# Autodesk Inventor assembly: Frame for Monitor Mounts Test
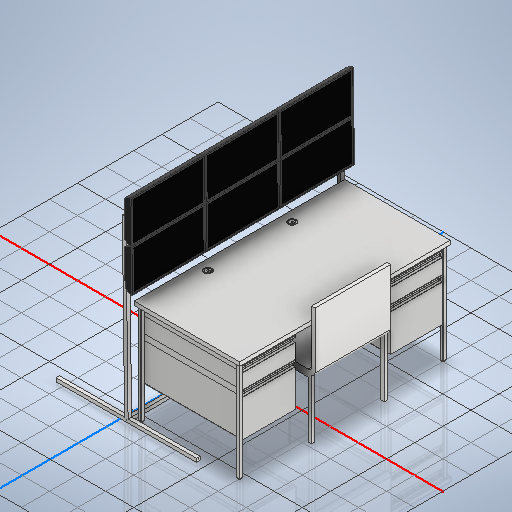
[picture p0: Inventor's stored thumbnail of the model, 512x512]
Saved by Autodesk Inventor 2027 (Build 310192000, 192)
## iProperties
Created: 2026-05-21
Part Number: Frame for Monitor Mounts Test
Document SubType Name: Assembly
Designer: IG2
Author: IG2
## Documents named in this file (8)
- C:\Users\ig2\Desktop\SMR Thermal\thermal-loop\resources\CAD_models\V0.1\Inventor\.iam files\Frame for Monitor Mounts Test.iam
- C:\Users\ig2\Downloads\Monitor v1.0.ipt
- C:\Users\ig2\Downloads\Monitor Base v1.0.ipt
- C:\Users\ig2\Downloads\Monitor Base Slide v1.0.ipt
- C:\Users\ig2\Downloads\Monitor Seat v1.0.ipt
- C:\Users\ig2\Desktop\SMR Thermal\thermal-loop\resources\CAD_models\V0.1\Inventor\.ipt files\Frame of Monitor Mount.ipt
- C:\Users\ig2\Desktop\SMR Thermal\thermal-loop\resources\CAD_models\V0.1\Inventor\.ipt files\chair.ipt
- C:\Users\ig2\Desktop\SMR Thermal\thermal-loop\resources\CAD_models\V0.1\Inventor\.ipt files\Plastic Laminate Top Desk Wide.ipt
## Components (27 placed, 7 different names)
1. Monitor v1.0:1 — Rigid:25, Rigid:32
2. Monitor v1.0:2 — Rigid:26, Rigid:29, Rigid:30
3. Monitor v1.0:3 — Rigid:24, Rigid:31, Rigid:32
4. Monitor v1.0:4 — Rigid:28, Rigid:31
5. Monitor v1.0:5 — Rigid:27, Rigid:29
6. Monitor v1.0:6 — Slider:19, Rigid:23, Rigid:30
7. Monitor Base v1.0:1 — Rotational:26
8. Monitor Base Slide v1.0:1 — Rigid:4, Rotational:26
9. Monitor Seat v1.0:1 — Rigid:1, Rigid:24, Rotational:33
10. Monitor Base v1.0:2 — Rigid:12
11. Monitor Base Slide v1.0:2 — Rigid:3, Rigid:12
12. Monitor Seat v1.0:2 — Rigid:3, Rigid:28
13. Monitor Base v1.0:3 — Rigid:2
14. Monitor Base Slide v1.0:3 — Rigid:1, Rigid:2
15. Monitor Seat v1.0:3 — Rigid:4, Rigid:25
16. Monitor Base v1.0:4 — Rigid:10
17. Monitor Base Slide v1.0:4 — Rigid:5, Rigid:10
18. Monitor Seat v1.0:4 — Rigid:5, Rigid:27
19. Monitor Base v1.0:5 — Rigid:9
20. Monitor Base Slide v1.0:5 — Rigid:6, Rigid:9
21. Monitor Seat v1.0:5 — Rigid:6, Slider:19, Rigid:23
22. Monitor Base v1.0:6 — Rigid:8
23. Monitor Base Slide v1.0:6 — Rigid:7, Rigid:8
24. Monitor Seat v1.0:6 — Rigid:7, Rigid:26, Rotational:32
25. Frame of Monitor Mount:1 — Rotational:32, Rotational:33
26. chair:1
27. Plastic Laminate Top Desk Wide:1
## Relationships (25: WeldJoint 21, RevoluteJoint 3, TranslationJoint 1)
- Rigid:1 [WeldJoint] (12.7 mm): Monitor Seat v1.0:1 ↔ Monitor Base Slide v1.0:3
- Rigid:2 [WeldJoint]: Monitor Base v1.0:3 ↔ Monitor Base Slide v1.0:3
- Rigid:3 [WeldJoint] (12.7 mm): Monitor Base Slide v1.0:2 ↔ Monitor Seat v1.0:2
- Rigid:4 [WeldJoint] (12.7 mm): Monitor Base Slide v1.0:1 ↔ Monitor Seat v1.0:3
- Rigid:5 [WeldJoint] (12.7 mm): Monitor Base Slide v1.0:4 ↔ Monitor Seat v1.0:4
- Rigid:6 [WeldJoint] (12.7 mm): Monitor Base Slide v1.0:5 ↔ Monitor Seat v1.0:5
- Rigid:7 [WeldJoint] (12.7 mm): Monitor Base Slide v1.0:6 ↔ Monitor Seat v1.0:6
- Rigid:8 [WeldJoint]: Monitor Base v1.0:6 ↔ Monitor Base Slide v1.0:6
- Rigid:9 [WeldJoint]: Monitor Base v1.0:5 ↔ Monitor Base Slide v1.0:5
- Rigid:10 [WeldJoint]: Monitor Base v1.0:4 ↔ Monitor Base Slide v1.0:4
- Rigid:12 [WeldJoint]: Monitor Base v1.0:2 ↔ Monitor Base Slide v1.0:2
- Slider:19 [TranslationJoint]: Monitor v1.0:6 ↔ Monitor Seat v1.0:5
- Rotational:26 [RevoluteJoint]: Monitor Base v1.0:1 ↔ Monitor Base Slide v1.0:1
- Rigid:23 [WeldJoint] (25.4 mm): Monitor v1.0:6 ↔ Monitor Seat v1.0:5
- Rigid:24 [WeldJoint] (25.4 mm): Monitor v1.0:3 ↔ Monitor Seat v1.0:1
- Rigid:25 [WeldJoint] (25.4 mm): Monitor v1.0:1 ↔ Monitor Seat v1.0:3
- Rigid:26 [WeldJoint] (25.4 mm): Monitor v1.0:2 ↔ Monitor Seat v1.0:6
- Rigid:27 [WeldJoint] (25.4 mm): Monitor v1.0:5 ↔ Monitor Seat v1.0:4
- Rigid:28 [WeldJoint] (25.4 mm): Monitor v1.0:4 ↔ Monitor Seat v1.0:2
- Rigid:29 [WeldJoint]: Monitor v1.0:2 ↔ Monitor v1.0:5
- Rigid:30 [WeldJoint]: Monitor v1.0:2 ↔ Monitor v1.0:6
- Rotational:32 [RevoluteJoint]: Monitor Seat v1.0:6 ↔ Frame of Monitor Mount:1
- Rigid:31 [WeldJoint]: Monitor v1.0:3 ↔ Monitor v1.0:4
- Rigid:32 [WeldJoint]: Monitor v1.0:1 ↔ Monitor v1.0:3
- Rotational:33 [RevoluteJoint]: Monitor Seat v1.0:1 ↔ Frame of Monitor Mount:1
